# Autodesk Inventor assembly: CLS_typeC_38.2N
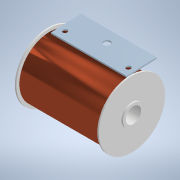
[picture p0: Inventor's stored thumbnail of the model, 180x180]
Saved by Autodesk Inventor 2021.3 (Build 253353010, 353A)
## iProperties
Created: 2021-06-04
Part Number: CLS_typeC_38.2N
Document SubType Name: Assembly
Designer: YusukeKunita
Author: YusukeKunita
## Documents named in this file (3)
- C:\Users\YusukeKunita\Documents\GrabCAD\NHK2021\BasicParts\よく使う部品（萩原）\ConstantLoadSpring\CLS_typeC_55.9N\CLS_typeC_55.9N.iam
- C:\Users\YusukeKunita\Documents\GrabCAD\NHK2021\BasicParts\よく使う部品（萩原）\ConstantLoadSpring\CLS_typeC_55.9N\CLS_typeC_55.9N_plate.ipt
- C:\Users\YusukeKunita\Documents\GrabCAD\NHK2021\BasicParts\よく使う部品（萩原）\ConstantLoadSpring\CLS_typeC_55.9N\CLS_typeC_55.9N.ipt
## Components (2 placed, 2 different names)
1. CLS_typeC_55.9N:1 — 正接:1, メイト:1, 正接:2
2. CLS_typeC_55.9N_plate:1 — 正接:1, メイト:1, 正接:2
## Relationships (3: Tangent 2, Mate 1)
- 正接:1 [Tangent]: CLS_typeC_55.9N:1 ↔ CLS_typeC_55.9N_plate:1
- メイト:1 [Mate] (1.8 mm): CLS_typeC_55.9N:1 ↔ CLS_typeC_55.9N_plate:1
- 正接:2 [Tangent]: CLS_typeC_55.9N:1 ↔ CLS_typeC_55.9N_plate:1
